# Autodesk Inventor assembly: field_with_robots
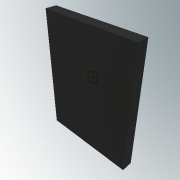
[picture p0: Inventor's stored thumbnail of the model, 180x180]
Saved by Autodesk Inventor 2020 (Build 240168000, 168)
## iProperties
Created: 2024-02-27
Part Number: field_with_robots
Document SubType Name: Assembly
Designer: 4s
Author: 4s
## Documents named in this file (3)
- C:\Users\4s\Documents\Inventor models\Asterisk\robot_v2\field_with_robots.iam
- C:\Users\4s\Documents\Inventor models\Asterisk\field.ipt
- C:\Users\4s\Documents\Inventor models\Asterisk\robot_v2\main2.iam
## Components (3 placed, 2 different names)
1. field:1 — Заподлицо:1, Совмещение:1, Заподлицо:2, Совмещение:2, Совмещение:3, Совмещение:4, Угол:1
2. main2:1 [sub-assembly] — Совмещение:3, Угол:2
3. main2:2 [sub-assembly] — Совмещение:4, Угол:1
## Relationships (8: Mate 4, Flush 2, Angle 2)
- Заподлицо:1 [Flush]: field:1
- Совмещение:1 [Mate]: field:1
- Заподлицо:2 [Flush]: field:1
- Совмещение:2 [Mate]: field:1
- Совмещение:3 [Mate] (9 mm): field:1 ↔ main2:1
- Совмещение:4 [Mate] (9 mm): field:1 ↔ main2:2
- Угол:1 [Angle] (70 deg): field:1 ↔ main2:2
- Угол:2 [Angle] (180 deg): main2:1
